# Autodesk Inventor assembly: II
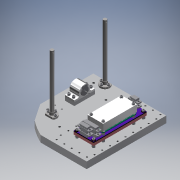
[picture p0: Inventor's stored thumbnail of the model, 180x180]
Saved by Autodesk Inventor 2017 (Build 210142000, 142)
## iProperties
Created: 2016-12-06
Part Number: II
Document SubType Name: Assembly
Designer: qupec
Mass: 1513.48 g
Surface Area: 2866.97 cm^2
Volume: 582.995 cm^3
Density: 2.59604 g/cm^3
Author: qupec
## Documents named in this file (19)
- C:\UMD\BPP\ROCKSAT X\STAR\CAD\Mechanical\Exploded Views\II.iam
- C:\UMD\BPP\ROCKSAT X\STAR\CAD\Mechanical\Full payload assembly\Subsystems\Slide Rods\Slide rod assembly.iam
- C:\UMD\BPP\ROCKSAT X\STAR\CAD\Mechanical\Full payload assembly\Subsystems\Electronics\Electronics Stack.iam
- C:\UMD\BPP\ROCKSAT X\STAR\CAD\Mechanical\Full payload assembly\Base Plate.ipt
- C:\UMD\BPP\ROCKSAT X\STAR\CAD\Mechanical\Full payload assembly\Subsystems\Shaker\ShakerAssembly.iam
- C:\UMD\BPP\ROCKSAT X\STAR\CAD\Mechanical\Full payload assembly\Subsystems\Fasteners\Num10 Belville Washer.ipt
- C:\UMD\BPP\ROCKSAT X\STAR\CAD\Mechanical\Full payload assembly\Subsystems\Fasteners\10-32 .375in Low Profile Socket Screw.ipt
- C:\UMD\BPP\ROCKSAT X\star\CAD\Mechanical\Subsystems\Full payload assembly mk 2\AIP\FEA\c3occb59c.fins
- C:\UMD\BPP\ROCKSAT X\star\CAD\Mechanical\Subsystems\Full payload assembly mk 2\AIP\FEA\c3occb5b4.fsat
- C:\UMD\BPP\ROCKSAT X\star\CAD\Mechanical\Subsystems\Full payload assembly mk 2\AIP\FEA\c3occb5b4.ftes
- C:\UMD\BPP\ROCKSAT X\star\CAD\Mechanical\Subsystems\Full payload assembly mk 2\AIP\FEA\c3occb5b4.fwiz
- C:\UMD\BPP\ROCKSAT X\star\CAD\Mechanical\Subsystems\Full payload assembly mk 2\AIP\FEA\c3occb5c0.fins
- C:\UMD\BPP\ROCKSAT X\star\CAD\Mechanical\Subsystems\Full payload assembly mk 2\AIP\FEA\c3occb5c0.fsat
- C:\UMD\BPP\ROCKSAT X\star\CAD\Mechanical\Subsystems\Full payload assembly mk 2\AIP\FEA\c3occb5c0.ftes
- C:\UMD\BPP\ROCKSAT X\star\CAD\Mechanical\Subsystems\Full payload assembly mk 2\AIP\FEA\c3occb5c0.fwiz
- C:\UMD\BPP\ROCKSAT X\star\CAD\Mechanical\Subsystems\Full payload assembly mk 2\AIP\FEA\c3occb60w.fmsh
- C:\UMD\BPP\ROCKSAT X\star\CAD\Mechanical\Subsystems\Full payload assembly mk 2\AIP\FEA\c3occb60x.fres
- C:\UMD\BPP\ROCKSAT X\star\CAD\Mechanical\Subsystems\Full payload assembly mk 2\AIP\FEA\c3occb6sg.fmsh
- C:\UMD\BPP\ROCKSAT X\star\CAD\Mechanical\Subsystems\Full payload assembly mk 2\AIP\FEA\c3occb6sh.fres
## Components (10 placed, 6 different names)
1. Slide rod assembly:1 [sub-assembly] — Mate:121
2. Electronics Stack:1 [sub-assembly] — Mate:397
3. Base Plate:1 — Mate:121, Mate:124, Flush:29, Flush:32, Mate:392, Mate:393, Mate:394, Mate:397
4. ShakerAssembly:1 [sub-assembly] — Mate:392, Mate:393, Mate:394
5. Num10 Belville Washer:1 — Mate:574
6. Num10 Belville Washer:3 — Mate:573
7. Num10 Belville Washer:4 — Mate:572
8. 10-32 .375in Low Profile Socket Screw:1 — Mate:574
9. 10-32 .375in Low Profile Socket Screw:2 — Mate:573
10. 10-32 .375in Low Profile Socket Screw:3 — Mate:572
## Relationships (11: Mate 9, Flush 2)
- Mate:121: Slide rod assembly:1 ↔ Base Plate:1
- Mate:124: Base Plate:1
- Flush:29: Base Plate:1
- Flush:32: Base Plate:1
- Mate:392: Base Plate:1 ↔ ShakerAssembly:1
- Mate:393: Base Plate:1 ↔ ShakerAssembly:1
- Mate:394: Base Plate:1 ↔ ShakerAssembly:1
- Mate:397: Electronics Stack:1 ↔ Base Plate:1
- Mate:572: Num10 Belville Washer:4 ↔ 10-32 .375in Low Profile Socket Screw:3
- Mate:573: Num10 Belville Washer:3 ↔ 10-32 .375in Low Profile Socket Screw:2
- Mate:574: Num10 Belville Washer:1 ↔ 10-32 .375in Low Profile Socket Screw:1
## Named parameters: sa_3 = 0, sa_4 = 29260.8, sa_5 = 0, sa_6 = 6894.76
note: some values were not read from the file. Shown as the stored number, unit unknown: "sa_3", "sa_4", "sa_5", "sa_6".
